# Autodesk Inventor assembly: SwarmieMini
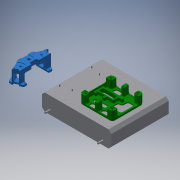
[picture p0: Inventor's stored thumbnail of the model, 180x180]
Saved by Autodesk Inventor 2016 (Build 200138000, 138)
## iProperties
Created: 2015-09-02
Part Number: SwarmieMini
Document SubType Name: Assembly
Designer: lachesis
Author: lachesis
## Documents named in this file (4)
- C:\Users\lachesis\git\Swarmie-Build\SwarmieMini Assembly\SwarmieMini.iam
- C:\Users\lachesis\git\Swarmie-Build\SwarmieMini Assembly\Parts\Chassis.ipt
- C:\Users\lachesis\git\Swarmie-Build\SwarmieMini Assembly\Parts\NUCBase-M.ipt
- C:\Users\lachesis\git\Swarmie-Build\SwarmieMini Assembly\Parts\USTowerLW-M.ipt
## Components (3 placed, 3 different names)
1. Chassis:1 — Mate:1, Mate:2, Mate:3, Mate:4, Mate:8
2. NUCBase-M:1
3. USTowerLW-M:1 — Mate:8
## Relationships (5: Mate 5)
- Mate:1: Chassis:1
- Mate:2: Chassis:1
- Mate:3: Chassis:1
- Mate:4: Chassis:1
- Mate:8: Chassis:1 ↔ USTowerLW-M:1
